# Autodesk Inventor assembly: AR-100
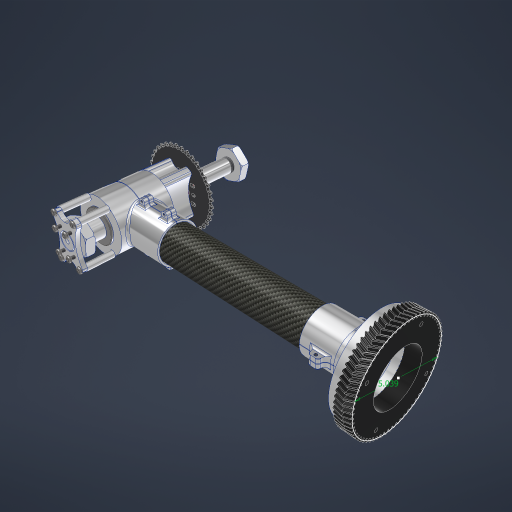
[picture p0: Inventor's stored thumbnail of the model, 512x512]
Saved by Autodesk Inventor 2023.4 (Build 274418000, 418)
## iProperties
Created: 2025-01-22
Part Number: AR-100
Document SubType Name: Assembly
Designer: slick
Mass: 6304.79 g
Surface Area: 14171.1 cm^2
Volume: 2619.67 cm^3
Density: 2.40671 g/cm^3
Author: slick
## Documents named in this file (23)
- C:\Users\brand\OneDrive\Documents\GitHub\robotics 23\2025-ReefScape---CAD\Arm\AR-100.iam
- C:\Users\brand\OneDrive\Documents\GitHub\robotics 23\2025-ReefScape---CAD\Arm\AR-001.ipt
- C:\Users\brand\OneDrive\Documents\GitHub\robotics 23\2025-ReefScape---CAD\COMMON PARTS\BEARINGS\0_875_ID_x_1_875_OD_X_0_500_Radial_Bearing_EE11S-2RS.ipt
- C:\Users\brand\OneDrive\Documents\GitHub\robotics 23\2025-ReefScape---CAD\Arm\AR-005.ipt
- C:\Users\brand\OneDrive\Documents\GitHub\robotics 23\2025-ReefScape---CAD\Arm\AR-006.ipt
- C:\Users\brand\OneDrive\Documents\GitHub\robotics 23\2025-ReefScape---CAD\COMMON PARTS\SPROCKETS\35\WCP-0983\WCP-0983.ipt
- C:\Users\brand\OneDrive\Documents\GitHub\robotics 23\2025-ReefScape---CAD\Arm\AR-009.ipt
- C:\Users\brand\OneDrive\Documents\GitHub\robotics 23\2025-ReefScape---CAD\Arm\AR-010.ipt
- C:\Users\brand\OneDrive\Documents\GitHub\robotics 23\2025-ReefScape---CAD\Arm\AR-013.ipt
- C:\Users\brand\OneDrive\Documents\GitHub\robotics 23\2025-ReefScape---CAD\Arm\AR-014.ipt
- C:\Users\brand\OneDrive\Documents\GitHub\robotics 23\2025-ReefScape---CAD\Elevator\EL2\EL2-A-012.ipt
- C:\Users\brand\OneDrive\Documents\GitHub\robotics 23\2025-ReefScape---CAD\Arm\AR-015.ipt
- C:\Users\brand\OneDrive\Documents\GitHub\robotics 23\2025-ReefScape---CAD\COMMON PARTS\SDS MK4i Swerve Module, 10-32, Falcons\CANcoder Assembly.iam
- C:\Users\brand\OneDrive\Documents\GitHub\robotics 23\2025-ReefScape---CAD\Content Center\en-US\U UNC 2605\Unbrako - 10 x 1 - 24(10).ipt
- C:\Users\brand\OneDrive\Documents\GitHub\robotics 23\2025-ReefScape---CAD\Content Center\en-US\U UNC 2605\Unbrako - 10 x 5_16 - 24(10).ipt
- C:\Users\brand\OneDrive\Documents\GitHub\robotics 23\2025-ReefScape---CAD\Content Center\en-US\U UNC 2605\Unbrako - 10 x 3_8 - 24(10).ipt
- C:\Users\brand\OneDrive\Documents\GitHub\robotics 23\2025-ReefScape---CAD\Gripper\GP5\GP5-300.iam
- C:\Users\brand\OneDrive\Documents\GitHub\robotics 23\2025-ReefScape---CAD\Arm\AR-016.ipt
- C:\Users\brand\OneDrive\Documents\GitHub\robotics 23\2025-ReefScape---CAD\Arm\AR-017.ipt
- C:\Users\brand\OneDrive\Documents\GitHub\robotics 23\2025-ReefScape---CAD\Arm\AR-018.ipt
- C:\Users\brand\OneDrive\Documents\GitHub\robotics 23\2025-ReefScape---CAD\Gripper\GP6\GP6-004.ipt
- C:\Users\brand\OneDrive\Documents\GitHub\robotics 23\2025-ReefScape---CAD\COMMON PARTS\4in Lazy Suzan.iam
- C:\Users\brand\OneDrive\Documents\GitHub\robotics 23\2025-ReefScape---CAD\COMMON PARTS\GEARS\Herringbone\2m 64t herringbone\2m 64t herringbone.ipt
## Components (42 placed, 22 different names)
1. AR-001:1 — Mate:1, Mate:2, Mate:3, Mate:4, Mate:13, Mate:14, Insert:37, Insert:38, Insert:39, Insert:40, Insert:92
2. 0_875_ID_x_1_875_OD_X_0_500_Radial_Bearing_EE11S-2RS:1 — Mate:1, Mate:3, Mate:15, Flush:2, Mate:20, Mate:25
3. 0_875_ID_x_1_875_OD_X_0_500_Radial_Bearing_EE11S-2RS:2 — Mate:2, Mate:4
4. AR-005:1 — Mate:13, Mate:14, Mate:17, Mate:18, Insert:92
5. AR-006:1 — Mate:15, Flush:2, Insert:36, Mate:19, Mate:21, Mate:22, Mate:24, Mate:26, Mate:28
6. WCP-0983:1 — Insert:21, Insert:22, Insert:23, Insert:24, Insert:45, Insert:46, Insert:47, Insert:48, Flush:4, Mate:27
7. AR-009:1 — Insert:21, Insert:22, Insert:23, Insert:24, Insert:39, Insert:40
8. AR-010:1 — Mate:17, Mate:18, Insert:93, Insert:94, Angle:1, Insert:99, Insert:100
9. AR-013:1 — Insert:36, Flush:7
10. AR-014:1 — Insert:37, Insert:38, Insert:41, Insert:42, Insert:49, Insert:50, Insert:51, Insert:52, Flush:5, Mate:22, Insert:95, Insert:96, Insert:97, Insert:98, Flush:7
11. EL2-A-012:1 — Mate:19, Mate:20, Flush:6, Mate:30
12. AR-015:1 — Insert:41, Insert:42, Insert:43, Insert:44, Insert:53, Insert:54, Insert:55, Insert:56
13. CANcoder Assembly:1 [sub-assembly] — Insert:43, Insert:44
14. GP5-300:1 [sub-assembly] — Insert:93, Insert:94
15. AR-016:1 — Insert:96
16. AR-016:2 — Insert:95
17. AR-016:3 — Insert:98
18. AR-016:4 — Insert:97
19. AR-017:1 — Mate:24, Mate:25, Mate:30
20. AR-018:1 — Mate:26, Mate:27, Angle:1
21. EL2-A-012:2 — Mate:28, Mate:29
22. GP6-004:1 — Insert:99, Insert:100, Insert:101, Insert:102
23. 4in Lazy Suzan:1 [sub-assembly] — Insert:101, Insert:102, Insert:103, Insert:104
24. 2m 64t herringbone:2 — Insert:103, Insert:104
25. Unbrako UNC Hex Socket Button Cap - Inch 10 x 1:1 — Insert:45
26. Unbrako UNC Hex Socket Button Cap - Inch 10 x 1:2 — Insert:46
27. Unbrako UNC Hex Socket Button Cap - Inch 10 x 1:3 — Insert:47
28. Unbrako UNC Hex Socket Button Cap - Inch 10 x 1:4 — Insert:48
29. Unbrako UNC Hex Socket Button Cap - Inch 10 x 1:5 — Insert:49
30. Unbrako UNC Hex Socket Button Cap - Inch 10 x 1:6 — Insert:50
31. Unbrako UNC Hex Socket Button Cap - Inch 10 x 1:7 — Insert:51
32. Unbrako UNC Hex Socket Button Cap - Inch 10 x 1:8 — Insert:52
33. Unbrako UNC Hex Socket Button Cap - Inch 10 x 5/16:1 — Insert:53
34. Unbrako UNC Hex Socket Button Cap - Inch 10 x 5/16:2 — Insert:54
35. Unbrako UNC Hex Socket Button Cap - Inch 10 x 5/16:3 — Insert:55
36. Unbrako UNC Hex Socket Button Cap - Inch 10 x 5/16:4 — Insert:56
37. Unbrako UNC Hex Socket Button Cap - Inch 10 x 3/8:16
38. Unbrako UNC Hex Socket Button Cap - Inch 10 x 3/8:17
39. Unbrako UNC Hex Socket Button Cap - Inch 10 x 3/8:18
40. Unbrako UNC Hex Socket Button Cap - Inch 10 x 3/8:25
41. Unbrako UNC Hex Socket Button Cap - Inch 10 x 3/8:26
42. Unbrako UNC Hex Socket Button Cap - Inch 10 x 3/8:27
## Relationships (64: Insert 38, Mate 20, Flush 5, Angle 1)
- Mate:1: AR-001:1 ↔ 0_875_ID_x_1_875_OD_X_0_500_Radial_Bearing_EE11S-2RS:1
- Mate:2: AR-001:1 ↔ 0_875_ID_x_1_875_OD_X_0_500_Radial_Bearing_EE11S-2RS:2
- Mate:3: AR-001:1 ↔ 0_875_ID_x_1_875_OD_X_0_500_Radial_Bearing_EE11S-2RS:1
- Mate:4: AR-001:1 ↔ 0_875_ID_x_1_875_OD_X_0_500_Radial_Bearing_EE11S-2RS:2
- Mate:13: AR-001:1 ↔ AR-005:1
- Mate:14 (-50.8 mm): AR-001:1 ↔ AR-005:1
- Mate:15: 0_875_ID_x_1_875_OD_X_0_500_Radial_Bearing_EE11S-2RS:1 ↔ AR-006:1
- Flush:2 (-12.7 mm): 0_875_ID_x_1_875_OD_X_0_500_Radial_Bearing_EE11S-2RS:1 ↔ AR-006:1
- Insert:21: WCP-0983:1 ↔ AR-009:1
- Insert:22: WCP-0983:1 ↔ AR-009:1
- Insert:23: WCP-0983:1 ↔ AR-009:1
- Insert:24: WCP-0983:1 ↔ AR-009:1
- Mate:17: AR-005:1 ↔ AR-010:1
- Mate:18: AR-005:1 ↔ AR-010:1
- Insert:36: AR-006:1 ↔ AR-013:1
- Insert:37: AR-001:1 ↔ AR-014:1
- Insert:38: AR-001:1 ↔ AR-014:1
- Insert:39: AR-001:1 ↔ AR-009:1
- Insert:40: AR-001:1 ↔ AR-009:1
- Mate:19: AR-006:1 ↔ EL2-A-012:1
- Mate:20: 0_875_ID_x_1_875_OD_X_0_500_Radial_Bearing_EE11S-2RS:1 ↔ EL2-A-012:1
- Insert:41: AR-014:1 ↔ AR-015:1
- Insert:42: AR-014:1 ↔ AR-015:1
- Insert:43: AR-015:1 ↔ CANcoder Assembly:1
- Insert:44: AR-015:1 ↔ CANcoder Assembly:1
- Insert:45: WCP-0983:1 ↔ Unbrako UNC Hex Socket Button Cap - Inch 10 x 1:1
- Insert:46: WCP-0983:1 ↔ Unbrako UNC Hex Socket Button Cap - Inch 10 x 1:2
- Insert:47: WCP-0983:1 ↔ Unbrako UNC Hex Socket Button Cap - Inch 10 x 1:3
- Insert:48: WCP-0983:1 ↔ Unbrako UNC Hex Socket Button Cap - Inch 10 x 1:4
- Insert:49: AR-014:1 ↔ Unbrako UNC Hex Socket Button Cap - Inch 10 x 1:5
- Insert:50: AR-014:1 ↔ Unbrako UNC Hex Socket Button Cap - Inch 10 x 1:6
- Insert:51: AR-014:1 ↔ Unbrako UNC Hex Socket Button Cap - Inch 10 x 1:7
- Insert:52: AR-014:1 ↔ Unbrako UNC Hex Socket Button Cap - Inch 10 x 1:8
- Insert:53: AR-015:1 ↔ Unbrako UNC Hex Socket Button Cap - Inch 10 x 5/16:1
- Insert:54: AR-015:1 ↔ Unbrako UNC Hex Socket Button Cap - Inch 10 x 5/16:2
- Insert:55: AR-015:1 ↔ Unbrako UNC Hex Socket Button Cap - Inch 10 x 5/16:3
- Insert:56: AR-015:1 ↔ Unbrako UNC Hex Socket Button Cap - Inch 10 x 5/16:4
- Insert:92: AR-001:1 ↔ AR-005:1
- Insert:93: AR-010:1 ↔ GP5-300:1
- Insert:94: AR-010:1 ↔ GP5-300:1
- Flush:4 (12.8307 mm): WCP-0983:1
- Mate:21 (-169.8625 mm): AR-006:1
- Flush:5: AR-014:1
- Mate:22: AR-006:1 ↔ AR-014:1
- Insert:95: AR-014:1 ↔ AR-016:2
- Insert:96: AR-014:1 ↔ AR-016:1
- Insert:97: AR-014:1 ↔ AR-016:4
- Insert:98: AR-014:1 ↔ AR-016:3
- Flush:6 (-10.9982 mm): EL2-A-012:1
- Mate:24: AR-006:1 ↔ AR-017:1
- Mate:25: 0_875_ID_x_1_875_OD_X_0_500_Radial_Bearing_EE11S-2RS:1 ↔ AR-017:1
- Mate:26: AR-006:1 ↔ AR-018:1
- Mate:27: WCP-0983:1 ↔ AR-018:1
- Mate:28: AR-006:1 ↔ EL2-A-012:2
- Mate:29 (63.5 mm): EL2-A-012:2
- Flush:7: AR-013:1 ↔ AR-014:1
- Mate:30: EL2-A-012:1 ↔ AR-017:1
- Angle:1 (0 deg): AR-010:1 ↔ AR-018:1
- Insert:99: AR-010:1 ↔ GP6-004:1
- Insert:100: AR-010:1 ↔ GP6-004:1
- Insert:101: GP6-004:1 ↔ 4in Lazy Suzan:1
- Insert:102: GP6-004:1 ↔ 4in Lazy Suzan:1
- Insert:103: 4in Lazy Suzan:1 ↔ 2m 64t herringbone:2
- Insert:104: 4in Lazy Suzan:1 ↔ 2m 64t herringbone:2
